# Autodesk Inventor assembly: MeasurementChamber - Assembly - Bade
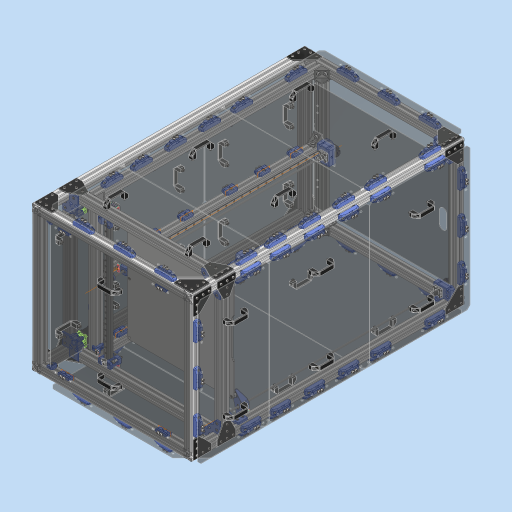
[picture p0: Inventor's stored thumbnail of the model, 512x512]
Saved by Autodesk Inventor 2023.2 (Build 272271000, 271)
## iProperties
Created: 2023-11-28
Part Number: MeasurementChamber - Assembly - Bade
Document SubType Name: Assembly
Designer: Nils Bade
Author: Nils Bade
## Documents named in this file (29)
- C:\Users\nilsb\Documents\Inventor\Projektarbeit-Bade\RatRig_Bade\MeasurementChamber - Assembly - Bade.iam
- C:\Users\nilsb\Documents\Inventor\Projektarbeit-Bade\RatRig_Bade\Z-Axis Transmission Assembly Back.iam
- C:\Users\nilsb\Documents\Inventor\Projektarbeit-Bade\RatRig_Bade\Z-Axis Transmission Assembly Front.iam
- C:\Users\nilsb\Documents\Inventor\Projektarbeit-Bade\RatRig_modified\Lead Screw - TR8x8-2p 1057mm Simple.ipt
- C:\Users\nilsb\Documents\Inventor\Projektarbeit-Bade\RatRig_modified\Leadscrew Constraint Front for 4040 - Assembly.iam
- C:\Users\nilsb\Documents\Inventor\Projektarbeit-Bade\RatRig_modified\Leadscrew Constraint Rear for 4040 - Assembly.iam
- C:\Users\nilsb\Documents\Inventor\Projektarbeit-Bade\RatRig_Bade\Bed Arm Back for 4040 - Assembly.iam
- C:\Users\nilsb\Documents\Inventor\Projektarbeit-Bade\RatRig_Bade\Bed Arm Left for 4040 - Assembly.iam
- C:\Users\nilsb\Documents\Inventor\Projektarbeit-Bade\RatRig_Bade\Bed Arm Right for 4040 - Assembly.iam
- C:\Users\nilsb\Documents\Inventor\Projektarbeit-Bade\RatRig_Bade\CoreXY Idler 4040 Assembly Left.iam
- C:\Users\nilsb\Documents\Inventor\Projektarbeit-Bade\RatRig_Bade\CoreXY Idler 4040 Assembly Right.iam
- C:\Users\nilsb\Documents\Inventor\Projektarbeit-Bade\RatRig_Bade\CoreXY Motor Assembly Left for 4040.iam
- C:\Users\nilsb\Documents\Inventor\Projektarbeit-Bade\RatRig_Bade\CoreXY Motor Assembly Right for 4040.iam
- C:\Users\nilsb\Documents\Inventor\Projektarbeit-Bade\RatRig_Bade\y-Max Endstop for 4040 - Assembly.iam
- C:\Users\nilsb\Documents\Inventor\Projektarbeit-Bade\RatRig_Bade\X-Gantry Assembly for 4040.iam
- C:\Users\nilsb\Documents\Inventor\Projektarbeit-Bade\RatRig_Bade\MeasurementChamber Frame Assembly - Bade v2.iam
- MeasurementChamber Frame Assembly - Bade v1.iam
- C:\Users\nilsb\Documents\Inventor\Projektarbeit-Bade\Enclosure\enc-SidePanel Unten - Assembly no Absorber.iam
- C:\Users\nilsb\Documents\Inventor\Projektarbeit-Bade\Enclosure\enc-SidePanel Mitte - Assembly no Absorber.iam
- C:\Users\nilsb\Documents\Inventor\Projektarbeit-Bade\Enclosure\enc-SidePanel Oben Links - Assembly no Absorber.iam
- C:\Users\nilsb\Documents\Inventor\Projektarbeit-Bade\Enclosure\enc-SidePanel Oben Rechts - Assembly no Absorber.iam
- C:\Users\nilsb\Documents\Inventor\Projektarbeit-Bade\Enclosure\enc-FrontPanel Oben - Assembly no Absorber.iam
- C:\Users\nilsb\Documents\Inventor\Projektarbeit-Bade\Enclosure\enc-TopPanel - Assembly no Absorber.iam
- C:\Users\nilsb\Documents\Inventor\Projektarbeit-Bade\Enclosure\enc-BackPanel Top - Assembly.iam
- C:\Users\nilsb\Documents\Inventor\Projektarbeit-Bade\Enclosure\enc-BackPanel Unten - Assembly.iam
- C:\Users\nilsb\Documents\Inventor\Projektarbeit-Bade\Enclosure\enc-BackPanel MitteRechts - Assembly.iam
- C:\Users\nilsb\Documents\Inventor\Projektarbeit-Bade\Enclosure\enc-BackPanel MitteLinks - Assembly.iam
- C:\Users\nilsb\Documents\Inventor\Projektarbeit-Bade\Enclosure\enc-BottomPanel.ipt
- C:\Users\nilsb\Documents\Inventor\Projektarbeit-Bade\RatRig_Bade\RatRig-Bade-BedAssembly.iam
## Components (36 placed, 26 different names)
1. MeasurementChamber Frame Assembly - Bade v1:2 [sub-assembly] — Passend:31, Passend:36, Passend:37, Passend:39, Passend:40, Fluchtend:32, Fluchtend:33, Passend:46, Fluchtend:34, Passend:48, Fluchtend:35, Fluchtend:36, Passend:49, Fluchtend:37, Fluchtend:38, Passend:50, Fluchtend:39, Passend:52, Fluchtend:40, Fluchtend:41, Passend:53, Fluchtend:42, Fluchtend:43, Fluchtend:44, Passend:55, Passend:56, Fluchtend:45, Fluchtend:46, Passend:57, Passend:58, Passend:59, Fluchtend:47, Passend:60, Fluchtend:62, Passend:61, Passend:62, Passend:63, Passend:64, Passend:65, Passend:66, Passend:67, Passend:68, Passend:69, Passend:70, Passend:71, Passend:72, Passend:73, Passend:74, Passend:75, Passend:76, Fluchtend:78, Passend:77, Fluchtend:79, Fluchtend:80
2. Z-Axis Transmission Assembly Back:1 [sub-assembly] — Passend:13
3. Z-Axis Transmission Assembly Front:1 [sub-assembly] — Passend:15
4. Z-Axis Transmission Assembly Front:2 [sub-assembly] — Passend:14
5. LeadScrew - TR8x8-2p 1057mm Simple:1 — Passend:13
6. LeadScrew - TR8x8-2p 1057mm Simple:2 — Passend:15
7. LeadScrew - TR8x8-2p 1057mm Simple:3 — Passend:14
8. Leadscrew Constraint Front for 4040 - Assembly:1 [sub-assembly] — Fluchtend:22, Fluchtend:1
9. Leadscrew Constraint Front for 4040 - Assembly:2 [sub-assembly] — Fluchtend:22
10. Leadscrew Constraint Rear for 4040 - Assembly:1 [sub-assembly] — Fluchtend:1
11. Bed Arm Back for 4040 - Assembly:1 [sub-assembly] — Fluchtend:29
12. Bed Arm Left for 4040 - Assembly:1 [sub-assembly] — Fluchtend:24, Fluchtend:29
13. Bed Arm Right for 4040 - Assembly:1 [sub-assembly] — Fluchtend:24, Passend:78
14. CoreXY Idler 4040 Assembly Left:1 [sub-assembly] — Passend:31
15. CoreXY Idler 4040 Assembly Right:1 [sub-assembly]
16. CoreXY Motor Assembly Left for 4040:1 [sub-assembly] — Passend:36, Passend:37
17. CoreXY Motor Assembly Right for 4040:1 [sub-assembly] — Passend:39, Passend:40
18. y-Max Endstop for 4040 - Assembly:1 [sub-assembly]
19. X-Gantry Assembly for 4040:1 [sub-assembly]
20. enc-SidePanel Unten - Assembly no Absorber:1 [sub-assembly] — Fluchtend:32, Fluchtend:33, Passend:46
21. enc-SidePanel Mitte - Assembly no Absorber:1 [sub-assembly] — Fluchtend:34, Passend:47, Passend:48
22. enc-SidePanel Oben Links - Assembly no Absorber:1 [sub-assembly] — Fluchtend:35, Fluchtend:36, Passend:49
23. enc-SidePanel Unten - Assembly no Absorber:2 [sub-assembly] — Fluchtend:37, Fluchtend:38, Passend:50, Passend:51
24. enc-SidePanel Mitte - Assembly no Absorber:2 [sub-assembly] — Fluchtend:39, Passend:51, Passend:52
25. enc-SidePanel Oben Links- Assembly no Absorber:1 [sub-assembly] — Fluchtend:40, Fluchtend:41, Passend:53
26. enc-SidePanel Unten - Assembly no Absorber:3 [sub-assembly] — Fluchtend:42, Fluchtend:43, Passend:54, Passend:56
27. enc-SidePanel Mitte - Assembly no Absorber:3 [sub-assembly] — Fluchtend:44, Passend:54, Passend:55
28. enc-SidePanel Oben Links - Assembly no Absorber:2 [sub-assembly] — Fluchtend:45, Fluchtend:46, Passend:57
29. enc-TopPanel - Assembly no Absorber:1 [sub-assembly] — Passend:58, Passend:59, Fluchtend:47, Passend:60
30. enc-BackPanel Top - Assembly:1 [sub-assembly] — Fluchtend:62, Passend:61, Passend:62, Passend:63
31. enc-BackPanel Unten - Assembly:1 [sub-assembly] — Passend:64, Passend:65, Passend:72
32. enc-BackPanel Unten - Assembly:2 [sub-assembly] — Passend:66, Passend:67, Passend:73
33. enc-BackPanel MitteRechts- Assembly:1 [sub-assembly] — Passend:70, Passend:71, Passend:74
34. enc-BackPanel MitteLinks - Assembly:1 [sub-assembly] — Passend:68, Passend:69, Passend:75
35. enc-BottomPanel:1 — Passend:76, Fluchtend:78, Passend:77
36. RatRig-Bade-BedAssembly:1 [sub-assembly] — Fluchtend:79, Passend:78, Fluchtend:80
## Relationships (106: Mate 77, Flush 29)
- [Mate]: MeasurementChamber Frame Assembly - Bade v1:2 ↔ Z-Axis Transmission Assembly Back:1
- [Mate]: MeasurementChamber Frame Assembly - Bade v1:2 ↔ Z-Axis Transmission Assembly Back:1
- [Mate]: MeasurementChamber Frame Assembly - Bade v1:2 ↔ Z-Axis Transmission Assembly Back:1
- [Mate]: MeasurementChamber Frame Assembly - Bade v1:2 ↔ Z-Axis Transmission Assembly Front:1
- [Mate]: MeasurementChamber Frame Assembly - Bade v1:2 ↔ Z-Axis Transmission Assembly Front:2
- [Mate]: MeasurementChamber Frame Assembly - Bade v1:2 ↔ Z-Axis Transmission Assembly Front:2
- [Mate]: MeasurementChamber Frame Assembly - Bade v1:2 ↔ Z-Axis Transmission Assembly Front:2
- [Mate]: MeasurementChamber Frame Assembly - Bade v1:2 ↔ Z-Axis Transmission Assembly Front:1
- [Mate]: MeasurementChamber Frame Assembly - Bade v1:2 ↔ Z-Axis Transmission Assembly Front:1
- [Mate]: MeasurementChamber Frame Assembly - Bade v1:2 ↔ LeadScrew - TR8x8-2p 1057mm Simple:1
- [Mate]: MeasurementChamber Frame Assembly - Bade v1:2 ↔ LeadScrew - TR8x8-2p 1057mm Simple:2
- [Mate]: MeasurementChamber Frame Assembly - Bade v1:2 ↔ LeadScrew - TR8x8-2p 1057mm Simple:3
- Passend:13 [Mate] (-10 mm): Z-Axis Transmission Assembly Back:1 ↔ LeadScrew - TR8x8-2p 1057mm Simple:1
- Passend:14 [Mate] (-10 mm): Z-Axis Transmission Assembly Front:2 ↔ LeadScrew - TR8x8-2p 1057mm Simple:3
- Passend:15 [Mate] (-10 mm): Z-Axis Transmission Assembly Front:1 ↔ LeadScrew - TR8x8-2p 1057mm Simple:2
- [Mate]: MeasurementChamber Frame Assembly - Bade v1:2 ↔ Leadscrew Constraint Front for 4040 - Assembly:2
- [Mate]: MeasurementChamber Frame Assembly - Bade v1:2 ↔ Leadscrew Constraint Front for 4040 - Assembly:2
- [Mate] (5 mm): MeasurementChamber Frame Assembly - Bade v1:2 ↔ Leadscrew Constraint Front for 4040 - Assembly:2
- [Mate]: MeasurementChamber Frame Assembly - Bade v1:2 ↔ Leadscrew Constraint Front for 4040 - Assembly:1
- [Mate]: MeasurementChamber Frame Assembly - Bade v1:2 ↔ Leadscrew Constraint Front for 4040 - Assembly:1
- Fluchtend:22 [Flush]: Leadscrew Constraint Front for 4040 - Assembly:1 ↔ Leadscrew Constraint Front for 4040 - Assembly:2
- [Mate]: MeasurementChamber Frame Assembly - Bade v1:2 ↔ Leadscrew Constraint Rear for 4040 - Assembly:1
- [Mate]: MeasurementChamber Frame Assembly - Bade v1:2 ↔ Leadscrew Constraint Rear for 4040 - Assembly:1
- Fluchtend:1 [Flush]: Leadscrew Constraint Front for 4040 - Assembly:1 ↔ Leadscrew Constraint Rear for 4040 - Assembly:1
- [Mate]: MeasurementChamber Frame Assembly - Bade v1:2 ↔ Bed Arm Back for 4040 - Assembly:1
- [Mate]: MeasurementChamber Frame Assembly - Bade v1:2 ↔ Bed Arm Back for 4040 - Assembly:1
- [Flush]: MeasurementChamber Frame Assembly - Bade v1:2 ↔ Bed Arm Left for 4040 - Assembly:1
- [Mate]: MeasurementChamber Frame Assembly - Bade v1:2 ↔ Bed Arm Left for 4040 - Assembly:1
- [Mate]: MeasurementChamber Frame Assembly - Bade v1:2 ↔ Bed Arm Right for 4040 - Assembly:1
- [Mate]: MeasurementChamber Frame Assembly - Bade v1:2 ↔ Bed Arm Right for 4040 - Assembly:1
- Fluchtend:24 [Flush]: Bed Arm Left for 4040 - Assembly:1 ↔ Bed Arm Right for 4040 - Assembly:1
- [Mate]: MeasurementChamber Frame Assembly - Bade v1:2 ↔ CoreXY Idler 4040 Assembly Left:1
- [Mate]: MeasurementChamber Frame Assembly - Bade v1:2 ↔ CoreXY Idler 4040 Assembly Left:1
- Passend:31 [Mate]: MeasurementChamber Frame Assembly - Bade v1:2 ↔ CoreXY Idler 4040 Assembly Left:1
- [Mate]: MeasurementChamber Frame Assembly - Bade v1:2 ↔ CoreXY Idler 4040 Assembly Right:1
- [Mate]: MeasurementChamber Frame Assembly - Bade v1:2 ↔ CoreXY Idler 4040 Assembly Right:1
- [Mate]: MeasurementChamber Frame Assembly - Bade v1:2 ↔ CoreXY Idler 4040 Assembly Right:1
- [Mate]: MeasurementChamber Frame Assembly - Bade v1:2 ↔ CoreXY Motor Assembly Left for 4040:1
- Passend:36 [Mate]: MeasurementChamber Frame Assembly - Bade v1:2 ↔ CoreXY Motor Assembly Left for 4040:1
- Passend:37 [Mate]: MeasurementChamber Frame Assembly - Bade v1:2 ↔ CoreXY Motor Assembly Left for 4040:1
- [Mate]: MeasurementChamber Frame Assembly - Bade v1:2 ↔ CoreXY Motor Assembly Right for 4040:1
- Passend:39 [Mate]: MeasurementChamber Frame Assembly - Bade v1:2 ↔ CoreXY Motor Assembly Right for 4040:1
- Passend:40 [Mate]: MeasurementChamber Frame Assembly - Bade v1:2 ↔ CoreXY Motor Assembly Right for 4040:1
- [Mate]: MeasurementChamber Frame Assembly - Bade v1:2 ↔ y-Max Endstop for 4040 - Assembly:1
- [Mate]: MeasurementChamber Frame Assembly - Bade v1:2 ↔ y-Max Endstop for 4040 - Assembly:1
- [Mate]: MeasurementChamber Frame Assembly - Bade v1:2 ↔ X-Gantry Assembly for 4040:1
- [Mate]: MeasurementChamber Frame Assembly - Bade v1:2 ↔ X-Gantry Assembly for 4040:1
- [Mate]: MeasurementChamber Frame Assembly - Bade v1:2 ↔ X-Gantry Assembly for 4040:1
- Fluchtend:26 [Flush] (135.5 mm)
- Fluchtend:28 [Flush] (1064.95 mm)
- Fluchtend:29 [Flush]: Bed Arm Back for 4040 - Assembly:1 ↔ Bed Arm Left for 4040 - Assembly:1
- Fluchtend:30 [Flush] (1000 mm)
- Fluchtend:31 [Flush] (500 mm)
- Fluchtend:32 [Flush]: MeasurementChamber Frame Assembly - Bade v1:2 ↔ enc-SidePanel Unten - Assembly no Absorber:1
- Fluchtend:33 [Flush]: MeasurementChamber Frame Assembly - Bade v1:2 ↔ enc-SidePanel Unten - Assembly no Absorber:1
- Passend:46 [Mate]: MeasurementChamber Frame Assembly - Bade v1:2 ↔ enc-SidePanel Unten - Assembly no Absorber:1
- Fluchtend:34 [Flush]: MeasurementChamber Frame Assembly - Bade v1:2 ↔ enc-SidePanel Mitte - Assembly no Absorber:1
- Passend:47 [Mate]: enc-SidePanel Mitte - Assembly no Absorber:1
- Passend:48 [Mate]: MeasurementChamber Frame Assembly - Bade v1:2 ↔ enc-SidePanel Mitte - Assembly no Absorber:1
- Fluchtend:35 [Flush]: MeasurementChamber Frame Assembly - Bade v1:2 ↔ enc-SidePanel Oben Links - Assembly no Absorber:1
- Fluchtend:36 [Flush]: MeasurementChamber Frame Assembly - Bade v1:2 ↔ enc-SidePanel Oben Links - Assembly no Absorber:1
- Passend:49 [Mate]: MeasurementChamber Frame Assembly - Bade v1:2 ↔ enc-SidePanel Oben Links - Assembly no Absorber:1
- Fluchtend:37 [Flush]: MeasurementChamber Frame Assembly - Bade v1:2 ↔ enc-SidePanel Unten - Assembly no Absorber:2
- Fluchtend:38 [Flush]: MeasurementChamber Frame Assembly - Bade v1:2 ↔ enc-SidePanel Unten - Assembly no Absorber:2
- Passend:50 [Mate]: MeasurementChamber Frame Assembly - Bade v1:2 ↔ enc-SidePanel Unten - Assembly no Absorber:2
- Fluchtend:39 [Flush]: MeasurementChamber Frame Assembly - Bade v1:2 ↔ enc-SidePanel Mitte - Assembly no Absorber:2
- Passend:51 [Mate]: enc-SidePanel Unten - Assembly no Absorber:2 ↔ enc-SidePanel Mitte - Assembly no Absorber:2
- Passend:52 [Mate]: MeasurementChamber Frame Assembly - Bade v1:2 ↔ enc-SidePanel Mitte - Assembly no Absorber:2
- Fluchtend:40 [Flush]: MeasurementChamber Frame Assembly - Bade v1:2 ↔ enc-SidePanel Oben Links- Assembly no Absorber:1
- Fluchtend:41 [Flush]: MeasurementChamber Frame Assembly - Bade v1:2 ↔ enc-SidePanel Oben Links- Assembly no Absorber:1
- Passend:53 [Mate]: MeasurementChamber Frame Assembly - Bade v1:2 ↔ enc-SidePanel Oben Links- Assembly no Absorber:1
- Fluchtend:42 [Flush]: MeasurementChamber Frame Assembly - Bade v1:2 ↔ enc-SidePanel Unten - Assembly no Absorber:3
- Fluchtend:43 [Flush]: MeasurementChamber Frame Assembly - Bade v1:2 ↔ enc-SidePanel Unten - Assembly no Absorber:3
- Fluchtend:44 [Flush]: MeasurementChamber Frame Assembly - Bade v1:2 ↔ enc-SidePanel Mitte - Assembly no Absorber:3
- Passend:54 [Mate]: enc-SidePanel Unten - Assembly no Absorber:3 ↔ enc-SidePanel Mitte - Assembly no Absorber:3
- Passend:55 [Mate]: MeasurementChamber Frame Assembly - Bade v1:2 ↔ enc-SidePanel Mitte - Assembly no Absorber:3
- Passend:56 [Mate]: MeasurementChamber Frame Assembly - Bade v1:2 ↔ enc-SidePanel Unten - Assembly no Absorber:3
- Fluchtend:45 [Flush]: MeasurementChamber Frame Assembly - Bade v1:2 ↔ enc-SidePanel Oben Links - Assembly no Absorber:2
- Fluchtend:46 [Flush]: MeasurementChamber Frame Assembly - Bade v1:2 ↔ enc-SidePanel Oben Links - Assembly no Absorber:2
- Passend:57 [Mate]: MeasurementChamber Frame Assembly - Bade v1:2 ↔ enc-SidePanel Oben Links - Assembly no Absorber:2
- Passend:58 [Mate]: MeasurementChamber Frame Assembly - Bade v1:2 ↔ enc-TopPanel - Assembly no Absorber:1
- Passend:59 [Mate]: MeasurementChamber Frame Assembly - Bade v1:2 ↔ enc-TopPanel - Assembly no Absorber:1
- Fluchtend:47 [Flush] (5 mm): MeasurementChamber Frame Assembly - Bade v1:2 ↔ enc-TopPanel - Assembly no Absorber:1
- Passend:60 [Mate]: MeasurementChamber Frame Assembly - Bade v1:2 ↔ enc-TopPanel - Assembly no Absorber:1
- Fluchtend:62 [Flush]: MeasurementChamber Frame Assembly - Bade v1:2 ↔ enc-BackPanel Top - Assembly:1
- Passend:61 [Mate]: MeasurementChamber Frame Assembly - Bade v1:2 ↔ enc-BackPanel Top - Assembly:1
- Passend:62 [Mate]: MeasurementChamber Frame Assembly - Bade v1:2 ↔ enc-BackPanel Top - Assembly:1
- Passend:63 [Mate]: MeasurementChamber Frame Assembly - Bade v1:2 ↔ enc-BackPanel Top - Assembly:1
- Passend:64 [Mate]: MeasurementChamber Frame Assembly - Bade v1:2 ↔ enc-BackPanel Unten - Assembly:1
- Passend:65 [Mate]: MeasurementChamber Frame Assembly - Bade v1:2 ↔ enc-BackPanel Unten - Assembly:1
- Passend:66 [Mate]: MeasurementChamber Frame Assembly - Bade v1:2 ↔ enc-BackPanel Unten - Assembly:2
- Passend:67 [Mate]: MeasurementChamber Frame Assembly - Bade v1:2 ↔ enc-BackPanel Unten - Assembly:2
- Passend:68 [Mate]: MeasurementChamber Frame Assembly - Bade v1:2 ↔ enc-BackPanel MitteLinks - Assembly:1
- Passend:69 [Mate]: MeasurementChamber Frame Assembly - Bade v1:2 ↔ enc-BackPanel MitteLinks - Assembly:1
- Passend:70 [Mate]: MeasurementChamber Frame Assembly - Bade v1:2 ↔ enc-BackPanel MitteRechts- Assembly:1
- Passend:71 [Mate]: MeasurementChamber Frame Assembly - Bade v1:2 ↔ enc-BackPanel MitteRechts- Assembly:1
- Passend:72 [Mate]: MeasurementChamber Frame Assembly - Bade v1:2 ↔ enc-BackPanel Unten - Assembly:1
- Passend:73 [Mate]: MeasurementChamber Frame Assembly - Bade v1:2 ↔ enc-BackPanel Unten - Assembly:2
- Passend:74 [Mate]: MeasurementChamber Frame Assembly - Bade v1:2 ↔ enc-BackPanel MitteRechts- Assembly:1
- Passend:75 [Mate]: MeasurementChamber Frame Assembly - Bade v1:2 ↔ enc-BackPanel MitteLinks - Assembly:1
- Passend:76 [Mate]: MeasurementChamber Frame Assembly - Bade v1:2 ↔ enc-BottomPanel:1
- Fluchtend:78 [Flush]: MeasurementChamber Frame Assembly - Bade v1:2 ↔ enc-BottomPanel:1
- Passend:77 [Mate]: MeasurementChamber Frame Assembly - Bade v1:2 ↔ enc-BottomPanel:1
- Fluchtend:79 [Flush]: MeasurementChamber Frame Assembly - Bade v1:2 ↔ RatRig-Bade-BedAssembly:1
- Passend:78 [Mate] (18 mm): Bed Arm Right for 4040 - Assembly:1 ↔ RatRig-Bade-BedAssembly:1
- Fluchtend:80 [Flush] (-327 mm): MeasurementChamber Frame Assembly - Bade v1:2 ↔ RatRig-Bade-BedAssembly:1
